# Autodesk Inventor assembly: 36T厚齿轮带铁芯
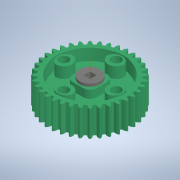
[picture p0: Inventor's stored thumbnail of the model, 180x180]
Saved by Autodesk Inventor 2020 (Build 240168000, 168)
## iProperties
Created: 2019-05-29
Part Number: 36T厚齿轮带铁芯
Document SubType Name: Assembly
Designer: aresp
Author: aresp
## Documents named in this file (3)
- C:\vault\ncrCadLib\齿轮\36T厚齿轮带铁芯.iam
- C:\vault\ncrCadLib\齿轮\Gear HS 36 tooth.ipt
- C:\vault\ncrCadLib\齿轮\Insert HS Metal.ipt
## Components (3 placed, 2 different names)
1. Gear HS 36 tooth:1 — 配合:2, 配合:3, 配合:4
2. Insert HS Metal:1 — 配合:1, 配合:2
3. Insert HS Metal:2 — 配合:1, 配合:3, 配合:4
## Relationships (4: Mate 4)
- 配合:1 [Mate]: Insert HS Metal:1 ↔ Insert HS Metal:2
- 配合:2 [Mate]: Gear HS 36 tooth:1 ↔ Insert HS Metal:1
- 配合:3 [Mate]: Gear HS 36 tooth:1 ↔ Insert HS Metal:2
- 配合:4 [Mate]: Gear HS 36 tooth:1 ↔ Insert HS Metal:2
